# Autodesk Inventor assembly: backmotors
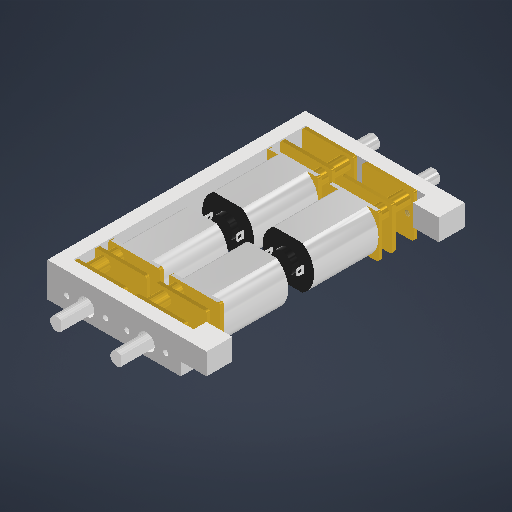
[picture p0: Inventor's stored thumbnail of the model, 512x512]
Saved by Autodesk Inventor 2026.2 (Build 302298010, 298A)
## iProperties
Created: 2026-04-27
Part Number: backmotors
Document SubType Name: Assembly
Designer: karol
Author: karol
## Documents named in this file (3)
- C:\Users\karol\Desktop\BOLT\cad\assembly\backmotors.iam
- C:\Users\karol\Desktop\BOLT\cad\ready parts\bmw.ipt
- C:\Users\karol\Desktop\BOLT\cad\ready parts\Pololu #2218 Micro Metal Gearmotor HP.ipt
## Components (5 placed, 2 different names)
1. bmw:1 — Zestawiające:1, Zestawiające:2, Zestawiające:3, Zestawiające:4, Zestawiające:5, Zestawiające:6, Zestawiające:7, Zestawiające:8, Zestawiające:9, Zestawiające:10, Zestawiające:11, Zestawiające:12, Zestawiające:13, Zestawiające:14
2. Pololu #2218 Micro Metal Gearmotor HP:1 — Zestawiające:5, Zestawiające:6, Zestawiające:12
3. Pololu #2218 Micro Metal Gearmotor HP:2 — Zestawiające:7, Zestawiające:8, Zestawiające:11, Zestawiające:13
4. Pololu #2218 Micro Metal Gearmotor HP:3 — Zestawiające:3, Zestawiające:4, Zestawiające:9
5. Pololu #2218 Micro Metal Gearmotor HP:4 — Zestawiające:1, Zestawiające:2, Zestawiające:10, Zestawiające:14
## Relationships (14: Mate 14)
- Zestawiające:1 [Mate]: bmw:1 ↔ Pololu #2218 Micro Metal Gearmotor HP:4
- Zestawiające:2 [Mate]: bmw:1 ↔ Pololu #2218 Micro Metal Gearmotor HP:4
- Zestawiające:3 [Mate]: bmw:1 ↔ Pololu #2218 Micro Metal Gearmotor HP:3
- Zestawiające:4 [Mate]: bmw:1 ↔ Pololu #2218 Micro Metal Gearmotor HP:3
- Zestawiające:5 [Mate]: bmw:1 ↔ Pololu #2218 Micro Metal Gearmotor HP:1
- Zestawiające:6 [Mate]: bmw:1 ↔ Pololu #2218 Micro Metal Gearmotor HP:1
- Zestawiające:7 [Mate]: bmw:1 ↔ Pololu #2218 Micro Metal Gearmotor HP:2
- Zestawiające:8 [Mate]: bmw:1 ↔ Pololu #2218 Micro Metal Gearmotor HP:2
- Zestawiające:9 [Mate]: bmw:1 ↔ Pololu #2218 Micro Metal Gearmotor HP:3
- Zestawiające:10 [Mate]: bmw:1 ↔ Pololu #2218 Micro Metal Gearmotor HP:4
- Zestawiające:11 [Mate]: bmw:1 ↔ Pololu #2218 Micro Metal Gearmotor HP:2
- Zestawiające:12 [Mate]: bmw:1 ↔ Pololu #2218 Micro Metal Gearmotor HP:1
- Zestawiające:13 [Mate]: bmw:1 ↔ Pololu #2218 Micro Metal Gearmotor HP:2
- Zestawiające:14 [Mate]: bmw:1 ↔ Pololu #2218 Micro Metal Gearmotor HP:4
